# Autodesk Inventor assembly: Assembled Horns
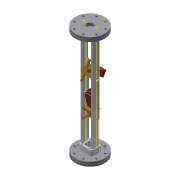
[picture p0: Inventor's stored thumbnail of the model, 180x180]
Saved by Autodesk Inventor 2015 (Build 190159000, 159)
## iProperties
Created: 2016-04-14
Part Number: Assembled Horns
Document SubType Name: Assembly
Designer: jad211
Author: jad211
## Documents named in this file (3)
- C:\CADFiles\EDM Machine\Detection Region\Microwave Horn Assembly\Assembled Horns.iam
- C:\CADFiles\EDM Machine\Detection Region\Microwave Horn Assembly\innerHorn slider.iam
- C:\CADFiles\EDM Machine\Detection Region\Microwave Horn Assembly\outerHorn slider.iam
## Components (2 placed, 2 different names)
1. innerHorn slider:1 [sub-assembly] — Mate:1, Angle:1, Mate:2
2. outerHorn slider:1 [sub-assembly] — Mate:1, Angle:1, Mate:2
## Relationships (3: Mate 2, Angle 1)
- Mate:1: innerHorn slider:1 ↔ outerHorn slider:1
- Angle:1 (0 deg): innerHorn slider:1 ↔ outerHorn slider:1
- Mate:2 (400 mm): innerHorn slider:1 ↔ outerHorn slider:1
